# Autodesk Inventor assembly: SAFRS-A-0010
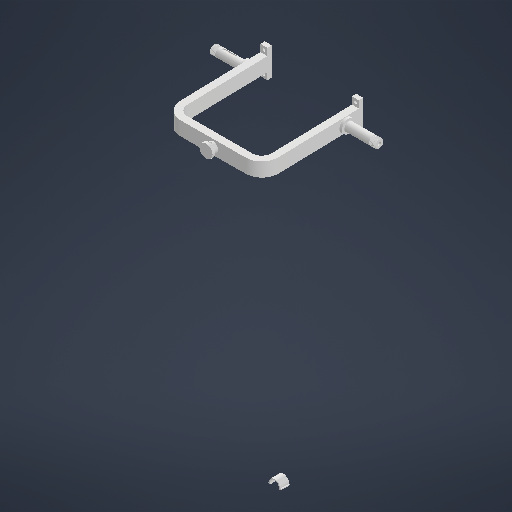
[picture p0: Inventor's stored thumbnail of the model, 512x512]
Saved by Autodesk Inventor 2026.2 (Build 302298000, 298)
## iProperties
Created: 2025-12-01
Part Number: SAFRS-A-0010
Document SubType Name: Assembly
Designer: jaewook
Author: jaewook
Title: Roll Support Rear v1 Assembly
## Documents named in this file (4)
- C:\Users\jk000\OneDrive\Desktop\git\SAFRS\mechanical\inventor\02__subassemblies\roll_support_rear_v1.iam
- C:\Users\jk000\OneDrive\Desktop\git\SAFRS\mechanical\inventor\01_parts\solid_6.ipt
- C:\Users\jk000\OneDrive\Desktop\git\SAFRS\mechanical\inventor\01_parts\stopper.ipt
- C:\Users\jk000\OneDrive\Desktop\git\SAFRS\mechanical\inventor\01_parts\rotation_stopper.ipt
## Components (3 placed, 3 different names)
1. solid_6:1 — 메이트:1, 메이트:2
2. stopper:1 — 메이트:1, 메이트:2
3. rotation_stopper:1
## Relationships (2: Mate 2)
- 메이트:1 [Mate]: solid_6:1 ↔ stopper:1
- 메이트:2 [Mate]: solid_6:1 ↔ stopper:1
